# Autodesk Inventor assembly: door_hinge_MIR
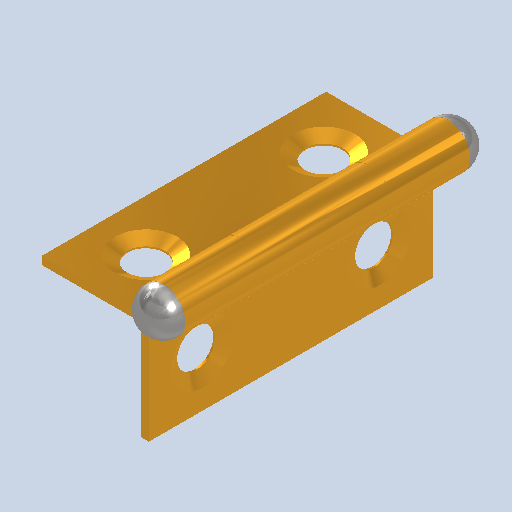
[picture p0: Inventor's stored thumbnail of the model, 512x512]
Saved by Autodesk Inventor 2023.2 (Build 272271030, 271C)
## iProperties
Created: 2022-08-13
Part Number: door_hinge_MIR
Document SubType Name: Assembly
Designer: I9232
Author: User
## Documents named in this file (4)
- D:\!project\fox_n_crow_construction\crow\face\door_hinge_MIR.iam
- D:\!project\fox_n_crow_construction\crow\face\hinge_component1_MIR.ipt
- D:\!project\fox_n_crow_construction\crow\face\hinge_axis_MIR.ipt
- D:\!project\fox_n_crow_construction\crow\face\hinge_component2_MIR.ipt
## Components (3 placed, 3 different names)
1. hinge_component1_MIR:1 — Заподлицо:2, Совмещение:2, Заподлицо:1
2. hinge_axis_MIR:1 — Заподлицо:2, Совмещение:2, Совмещение:1
3. hinge_component2_MIR:1 — Заподлицо:1, Совмещение:1
## Relationships (4: Flush 2, Mate 2)
- Заподлицо:2 [Flush]: hinge_component1_MIR:1 ↔ hinge_axis_MIR:1
- Совмещение:2 [Mate]: hinge_component1_MIR:1 ↔ hinge_axis_MIR:1
- Заподлицо:1 [Flush]: hinge_component1_MIR:1 ↔ hinge_component2_MIR:1
- Совмещение:1 [Mate]: hinge_axis_MIR:1 ↔ hinge_component2_MIR:1
